# Autodesk Inventor assembly: JointsMergedAssembly
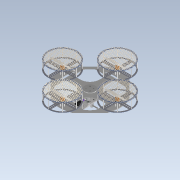
[picture p0: Inventor's stored thumbnail of the model, 180x180]
Saved by Autodesk Inventor 2021.1 (Build 251245010, 245A)
## iProperties
Created: 2024-03-10
Part Number: JointsMergedAssembly
Document SubType Name: Assembly
Designer: user
Author: user
## Documents named in this file (3)
- F:\College\Semester_10\GP2\2DOF\2DOF_Hover\CAD\Workspaces\Workspace\JointsMergedAssembly.iam
- F:\College\Semester_10\GP2\2DOF\2DOF_Hover\CAD\Workspaces\Workspace\SecondJoint.iam
- F:\College\Semester_10\GP2\2DOF\2DOF_Hover\CAD\Workspaces\Workspace\FirstJoint.iam
## Components (2 placed, 2 different names)
1. SecondJoint:1 [sub-assembly]
2. FirstJoint:1 [sub-assembly] — Mate:2, Mate:3, Mate:4
## Relationships (6: Mate 4, Flush 1, Angle 1)
- [Mate]: SecondJoint:1 ↔ FirstJoint:1
- [Flush] (-30 mm): SecondJoint:1 ↔ FirstJoint:1
- [Angle] (0 deg): SecondJoint:1 ↔ FirstJoint:1
- Mate:2 (-9 mm): FirstJoint:1
- Mate:3 (-24 mm): FirstJoint:1
- Mate:4: FirstJoint:1
